# Autodesk Inventor assembly: mozgasvizsgalat_mozgo
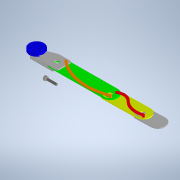
[picture p0: Inventor's stored thumbnail of the model, 180x180]
Saved by Autodesk Inventor 2020 (Build 240168000, 168)
## iProperties
Created: 2019-08-09
Part Number: mozgasvizsgalat_mozgo
Document SubType Name: Assembly
Designer: Horváth Patrik
Author: Horváth Patrik
## Documents named in this file (10)
- D:\I.V.A.N\LEGO\INDACT\Robotkéz\kéz12.0\Mozgásvizsgálat\mozgasvizsgalat_mozgo.iam
- D:\I.V.A.N\LEGO\INDACT\Robotkéz\kéz12.0\Mozgásvizsgálat\Solid1.ipt
- D:\I.V.A.N\LEGO\INDACT\Robotkéz\kéz12.0\Mozgásvizsgálat\Solid2.ipt
- D:\I.V.A.N\LEGO\INDACT\Robotkéz\kéz12.0\Mozgásvizsgálat\Solid3.ipt
- D:\I.V.A.N\LEGO\INDACT\Robotkéz\kéz12.0\Mozgásvizsgálat\Solid4.ipt
- D:\I.V.A.N\LEGO\INDACT\Robotkéz\kéz12.0\Mozgásvizsgálat\Solid5.ipt
- D:\I.V.A.N\LEGO\INDACT\Robotkéz\kéz12.0\Mozgásvizsgálat\Solid6.ipt
- D:\I.V.A.N\LEGO\INDACT\Robotkéz\kéz12.0\Mozgásvizsgálat\Solid7.ipt
- D:\I.V.A.N\LEGO\INDACT\Robotkéz\kéz12.0\Mozgásvizsgálat\Solid8.ipt
- C:\Users\Horváth Patrik\Documents\Inventor\Content Center Files\R2020\en-US\ISO 4762(2)\ISO 4762 - M2 x 10ISO.ipt
## Components (9 placed, 9 different names)
1. Solid1:1 — Mate:1, Mate:4, Mate:9, Mate:10, Mate:15, Flush:1
2. Solid2:1 — Mate:1, Mate:4, Mate:5, Mate:7, Mate:11, Mate:12, Mate:16, Mate:18
3. Solid3:1 — Mate:5, Mate:6, Mate:7, Mate:8, Mate:13, Flush:2
4. Solid4:1 — Mate:6, Mate:8, Mate:14, Flush:2
5. Solid5:1 — Mate:9, Mate:10, Mate:13
6. Solid6:1 — Mate:11, Mate:12, Mate:14
7. Solid7:1 — Mate:15, Flush:1, Mate:17
8. Solid8:1 — Mate:16, Mate:17, Mate:18
9. ISO 4762 M2 x 10:1
## Relationships (18: Mate 16, Flush 2)
- Mate:1: Solid1:1 ↔ Solid2:1
- Mate:4: Solid1:1 ↔ Solid2:1
- Mate:5: Solid2:1 ↔ Solid3:1
- Mate:6: Solid3:1 ↔ Solid4:1
- Mate:7: Solid2:1 ↔ Solid3:1
- Mate:8: Solid3:1 ↔ Solid4:1
- Mate:9: Solid1:1 ↔ Solid5:1
- Mate:10: Solid1:1 ↔ Solid5:1
- Mate:11: Solid2:1 ↔ Solid6:1
- Mate:12: Solid2:1 ↔ Solid6:1
- Mate:13: Solid3:1 ↔ Solid5:1
- Mate:14: Solid4:1 ↔ Solid6:1
- Mate:15: Solid1:1 ↔ Solid7:1
- Flush:1: Solid1:1 ↔ Solid7:1
- Mate:16: Solid2:1 ↔ Solid8:1
- Mate:17: Solid7:1 ↔ Solid8:1
- Mate:18: Solid2:1 ↔ Solid8:1
- Flush:2: Solid3:1 ↔ Solid4:1
